# Autodesk Inventor assembly: Anglerfish_VCM_v2
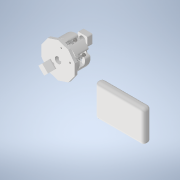
[picture p0: Inventor's stored thumbnail of the model, 180x180]
Saved by Autodesk Inventor 2022 (Build 260153000, 153)
## iProperties
Created: 2022-04-02
Part Number: Anglerfish_VCM_v2
Document SubType Name: Assembly
Designer: Prakash Lab
Author: Prakash Lab
## Documents named in this file (11)
- C:\Users\diederichbenedict\Dropbox\Dokumente\Promotion\PROJECTS\Matchboxscope\INVENTOR\Anglerfish_VCM_v2.iam
- C:\Users\diederichbenedict\Dropbox\Dokumente\Promotion\PROJECTS\Matchboxscope\INVENTOR\00_ESP3-CAM.iam
- C:\Users\diederichbenedict\Dropbox\Dokumente\Promotion\PROJECTS\Matchboxscope\INVENTOR\00_Powerbank.ipt
- C:\Users\diederichbenedict\Dropbox\Dokumente\Promotion\PROJECTS\Matchboxscope\INVENTOR\00_spring.ipt
- C:\Users\diederichbenedict\Documents\Inventor\Content Center Files\R2022\de-DE\DIN 912\DIN 912 - M3 x 0.5 x 25 x 18.ipt
- C:\Users\diederichbenedict\Dropbox\Dokumente\Promotion\PROJECTS\Matchboxscope\INVENTOR\00_bonne_maman_jar.ipt
- C:\Users\diederichbenedict\Dropbox\Dokumente\Promotion\PROJECTS\Matchboxscope\INVENTOR\Anglerfish_Jar_Adapterplate_v1.ipt
- C:\Users\diederichbenedict\Dropbox\Dokumente\Promotion\PROJECTS\Matchboxscope\INVENTOR\Anglerfish_Lightperiscope_long_V0.ipt
- C:\Users\diederichbenedict\Dropbox\Dokumente\Promotion\PROJECTS\Matchboxscope\INVENTOR\Anglerfish_bottom_v0.ipt
- C:\Users\diederichbenedict\Dropbox\Dokumente\Promotion\PROJECTS\Matchboxscope\INVENTOR\Anglerfish_middle2_m12VCMLens_v2.ipt
- C:\Users\diederichbenedict\Dropbox\Dokumente\Promotion\PROJECTS\Matchboxscope\INVENTOR\00_CCTV_M12_VCM.ipt
## Components (14 placed, 10 different names)
1. Anglerfish_middle2_m12VCMLens_v2:1 — Insert:1, Angle:1, Mate:5, Passend:6
2. Anglerfish_bottom_v0:1 — Mate:1, Mate:2, Mate:3, Mate:4, Flush:1, Mate:5
3. 00_ESP3-CAM:1 [sub-assembly] — Mate:4, Flush:1, Insert:1
4. Anglerfish_Jar_Adapterplate_v1:1 — Einfügen:12, Einfügen:13, Einfügen:14, Einfügen:15, Einfügen:16, Passend:6, Einfügen:17, Passend:7
5. 00_Powerbank:1
6. 00_spring:1 — Einfügen:16
7. 00_bonne_maman_jar:1 — Winkel:2, Passend:7
8. DIN 912 - ersetzt durch DIN EN ISO 4762 M3 x 25:5 — Einfügen:17
9. 00_spring:5 — Einfügen:15
10. DIN 912 - ersetzt durch DIN EN ISO 4762 M3 x 25:7 — Einfügen:12
11. 00_spring:6 — Einfügen:14
12. DIN 912 - ersetzt durch DIN EN ISO 4762 M3 x 25:8 — Einfügen:13
13. Anglerfish_Lightperiscope_long_V0:1
14. 00_CCTV_M12_VCM:1
## Relationships (17: Mate 7, Insert 7, Angle 2, Flush 1)
- Mate:1: Anglerfish_bottom_v0:1
- Mate:2: Anglerfish_bottom_v0:1
- Mate:3: Anglerfish_bottom_v0:1
- Mate:4: Anglerfish_bottom_v0:1 ↔ 00_ESP3-CAM:1
- Flush:1: Anglerfish_bottom_v0:1 ↔ 00_ESP3-CAM:1
- Insert:1: Anglerfish_middle2_m12VCMLens_v2:1 ↔ 00_ESP3-CAM:1
- Angle:1 (0 deg): Anglerfish_middle2_m12VCMLens_v2:1
- Mate:5: Anglerfish_middle2_m12VCMLens_v2:1 ↔ Anglerfish_bottom_v0:1
- Winkel:2 [Angle] (0 deg): 00_bonne_maman_jar:1
- Einfügen:12 [Insert]: Anglerfish_Jar_Adapterplate_v1:1 ↔ DIN 912 - ersetzt durch DIN EN ISO 4762 M3 x 25:7
- Einfügen:13 [Insert]: Anglerfish_Jar_Adapterplate_v1:1 ↔ DIN 912 - ersetzt durch DIN EN ISO 4762 M3 x 25:8
- Einfügen:14 [Insert]: Anglerfish_Jar_Adapterplate_v1:1 ↔ 00_spring:6
- Einfügen:15 [Insert]: Anglerfish_Jar_Adapterplate_v1:1 ↔ 00_spring:5
- Einfügen:16 [Insert]: Anglerfish_Jar_Adapterplate_v1:1 ↔ 00_spring:1
- Passend:6 [Mate] (5 mm): Anglerfish_middle2_m12VCMLens_v2:1 ↔ Anglerfish_Jar_Adapterplate_v1:1
- Einfügen:17 [Insert]: Anglerfish_Jar_Adapterplate_v1:1 ↔ DIN 912 - ersetzt durch DIN EN ISO 4762 M3 x 25:5
- Passend:7 [Mate]: Anglerfish_Jar_Adapterplate_v1:1 ↔ 00_bonne_maman_jar:1
